# Autodesk Inventor assembly: FE-00022
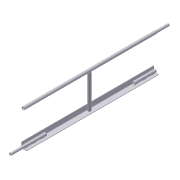
[picture p0: Inventor's stored thumbnail of the model, 180x180]
Saved by Autodesk Inventor 2012 (Build 160160000, 160)
## iProperties
Company: FIRST
Created: 2008-06-05
Part Number: FE-00022
Document SubType Name: Assembly
Designer: dfoster
Description: Field Rail Assy - Mid
Title: Field Rail Assy - Mid
Author: dfoster
## Documents named in this file (4)
- C:\Data Folder\FRC 2012 Field\Components\FE-00022.iam
- C:\Data Folder\FRC 2012 Field\Components\FE-00005.iam
- C:\Data Folder\FRC 2012 Field\Components\FE-00026.ipt
- C:\Data Folder\FRC 2012 Field\Components\HW-00010.ipt
## Components (7 placed, 3 different names)
1. FE-00005:1 [sub-assembly] — Mate:1, Angle:1, Flush:1, Mate:2, Angle:2, Flush:2, Tangent:1, Mate:4, Tangent:2
2. FE-00026:1 — Mate:1, Angle:1, Flush:1
3. FE-00026:2 — Mate:2, Angle:2, Flush:2
4. HW-00010:1 — Mate:4, Tangent:2
5. HW-00010:3
6. HW-00010:2 — Tangent:1
7. HW-00010:4
## Component patterns: (2 elements, first: HW-00010:1), (2 elements, first: HW-00010:2)
## Relationships (10: Mate 4, Angle 2, Flush 2, Tangent 2)
- Mate:1: FE-00005:1 ↔ FE-00026:1
- Angle:1 (0 deg): FE-00005:1 ↔ FE-00026:1
- Flush:1 (-177.8 mm): FE-00005:1 ↔ FE-00026:1
- Mate:2: FE-00005:1 ↔ FE-00026:2
- Angle:2 (0 deg): FE-00005:1 ↔ FE-00026:2
- Flush:2 (-177.8 mm): FE-00005:1 ↔ FE-00026:2
- [Mate]: FE-00005:1 ↔ HW-00010:2
- Tangent:1: FE-00005:1 ↔ HW-00010:2
- Mate:4: FE-00005:1 ↔ HW-00010:1
- Tangent:2: FE-00005:1 ↔ HW-00010:1
